# Autodesk Inventor assembly: compresor_completo
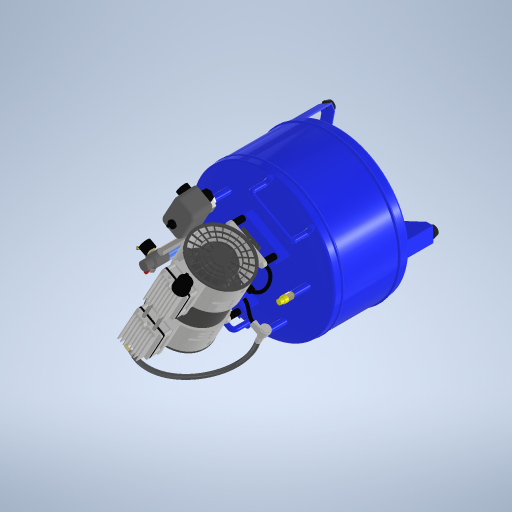
[picture p0: Inventor's stored thumbnail of the model, 512x512]
Saved by Autodesk Inventor 2024 (Build 280153000, 153)
## iProperties
Created: 2022-11-16
Part Number: compresor_completo
Document SubType Name: Assembly
Designer: ferna
Author: ferna
## Documents named in this file (11)
- C:\Users\ferna\OneDrive - Universidad Católica de Chile\Bocas\RobotFlautista\compresor_completo.iam
- C:\Users\ferna\OneDrive - Universidad Católica de Chile\Bocas\RobotFlautista\estanque.ipt
- C:\Users\ferna\OneDrive - Universidad Católica de Chile\Bocas\RobotFlautista\pata.ipt
- C:\Users\ferna\OneDrive - Universidad Católica de Chile\Bocas\RobotFlautista\salida_estanque.ipt
- C:\Users\ferna\OneDrive - Universidad Católica de Chile\Bocas\RobotFlautista\encendido.ipt
- C:\Users\ferna\OneDrive - Universidad Católica de Chile\Bocas\RobotFlautista\conector.ipt
- C:\Users\ferna\OneDrive - Universidad Católica de Chile\Bocas\RobotFlautista\valvula.ipt
- C:\Users\ferna\OneDrive - Universidad Católica de Chile\Bocas\RobotFlautista\motor.ipt
- C:\Users\ferna\OneDrive - Universidad Católica de Chile\Bocas\RobotFlautista\real_motor.ipt
- C:\Users\ferna\OneDrive - Universidad Católica de Chile\Bocas\RobotFlautista\compresor_completo.Harness1.iam
- C:\Users\ferna\OneDrive - Universidad Católica de Chile\Bocas\RobotFlautista\compresor_completo.Harness2.iam
## Components (12 placed, 10 different names)
1. estanque:1 — Mate:1, Mate:2, Mate:3, Mate:4, Mate:5, Mate:6, Mate:7, Mate:8, Mate:9, Angle:1, Mate:10, Mate:11, Mate:12, Mate:13, Mate:14, Mate:15, Angle:3, Mate:16, Mate:17, Flush:1, Mate:18, Mate:19, Mate:20
2. pata:1 — Mate:2, Mate:3
3. pata:2 — Mate:4, Mate:6
4. pata:3 — Mate:5, Mate:7
5. salida_estanque:1 — Mate:8, Mate:9, Angle:1, Angle:2
6. encendido:1 — Mate:10, Mate:11, Angle:2
7. conector:1 — Mate:12, Mate:15, Angle:3
8. valvula:1 — Mate:13, Mate:14
9. motor:1 — Mate:16, Mate:17, Flush:1
10. real_motor:1 — Mate:18, Mate:19, Mate:20
11. Harness1 [sub-assembly]
12. Harness2 [sub-assembly]
## Relationships (24: Mate 20, Angle 3, Flush 1)
- Mate:1: estanque:1
- Mate:2: estanque:1 ↔ pata:1
- Mate:3: estanque:1 ↔ pata:1
- Mate:4: estanque:1 ↔ pata:2
- Mate:5: estanque:1 ↔ pata:3
- Mate:6: estanque:1 ↔ pata:2
- Mate:7: estanque:1 ↔ pata:3
- Mate:8: estanque:1 ↔ salida_estanque:1
- Mate:9: estanque:1 ↔ salida_estanque:1
- Angle:1 (0 deg): estanque:1 ↔ salida_estanque:1
- Mate:10: estanque:1 ↔ encendido:1
- Mate:11: estanque:1 ↔ encendido:1
- Angle:2 (0 deg): salida_estanque:1 ↔ encendido:1
- Mate:12: estanque:1 ↔ conector:1
- Mate:13: estanque:1 ↔ valvula:1
- Mate:14: estanque:1 ↔ valvula:1
- Mate:15: estanque:1 ↔ conector:1
- Angle:3 (180 deg): estanque:1 ↔ conector:1
- Mate:16: estanque:1 ↔ motor:1
- Mate:17 (8.45 mm): estanque:1 ↔ motor:1
- Flush:1 (17.81 mm): estanque:1 ↔ motor:1
- Mate:18: estanque:1 ↔ real_motor:1
- Mate:19: estanque:1 ↔ real_motor:1
- Mate:20: estanque:1 ↔ real_motor:1
